# Autodesk Inventor assembly: full drive
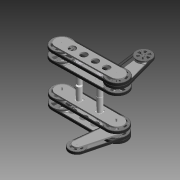
[picture p0: Inventor's stored thumbnail of the model, 180x180]
Saved by Autodesk Inventor 2011 (Build 150239000, 239)
## iProperties
Created: 2010-04-20
Part Number: full drive
Document SubType Name: Assembly
Designer: lucio
Mass: 6228.7 g
Surface Area: 18313.6 cm^2
Volume: 6152.03 cm^3
Density: 1.01246 g/cm^3
Author: lucio
## Documents named in this file (2)
- C:\Users\lucio\Documents\Inventor\caterpillar\full drive.iam
- C:\Users\lucio\Documents\Inventor\caterpillar\left drive.iam
## Components (2 placed, 1 different names)
1. left drive:1 [sub-assembly] — Mate:1, Mate:2, Mate:3
2. left drive:2 [sub-assembly] — Mate:1, Mate:2, Mate:3
## Relationships (3: Mate 3)
- Mate:1: left drive:1 ↔ left drive:2
- Mate:2: left drive:1 ↔ left drive:2
- Mate:3 (2 mm): left drive:1 ↔ left drive:2
